# Autodesk Inventor assembly: BUMP_000_Bumpers
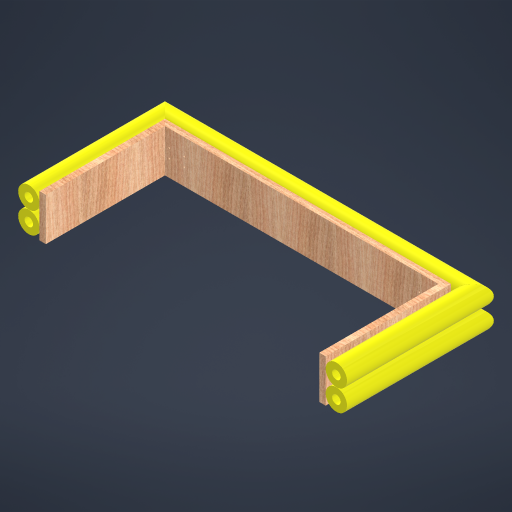
[picture p0: Inventor's stored thumbnail of the model, 512x512]
Saved by Autodesk Inventor 2024.2 (Build 282272000, 272)
## iProperties
Created: 2024-08-06
Part Number: BUMP_000_Bumpers
Document SubType Name: Assembly
Designer: Bryan
Mass: 492.361 g
Surface Area: 10037.4 cm^2
Volume: 9172.55 cm^3
Density: 0.0536776 g/cm^3
Author: Bryan
## Documents named in this file (8)
- C:\Users\bobsb\OneDrive\Documents\GitHub\1622-2024-Summer-CAD-A-Thon\Bumper\BUMP_000_Bumpers.iam
- C:\Users\bobsb\OneDrive\Documents\GitHub\1622-2024-Summer-CAD-A-Thon\Bumper\BUMP_001_Wood1.ipt
- C:\Users\bobsb\OneDrive\Documents\GitHub\1622-2024-Summer-CAD-A-Thon\Bumper\BUMP_002_Wood2.ipt
- C:\Users\bobsb\OneDrive\Documents\GitHub\1622-2024-Summer-CAD-A-Thon\COTS Library\Stucture\COTS_88805K219_Architectural 6063 Aluminum 90 Degree Angle.ipt
- C:\Users\bobsb\OneDrive\Documents\GitHub\1622-2024-Summer-CAD-A-Thon\COTS Library\Fasteners\Wood Screws\COTS_BumperWoodScrew_90031A197_Phillips Flat Head Screws for Wood.ipt
- C:\Users\bobsb\OneDrive\Documents\GitHub\1622-2024-Summer-CAD-A-Thon\Bumper\BUMP_003_Noodle1.ipt
- C:\Users\bobsb\OneDrive\Documents\GitHub\1622-2024-Summer-CAD-A-Thon\Bumper\BUMP_004_Noodle2.ipt
- C:\Users\bobsb\Downloads\th.jpg
## Components (27 placed, 6 different names)
1. BUMP_001_Wood1:1 — Mate:5, Mate:6, Flush:3, Mate:28, Mate:29, Flush:4, Mate:30, Mate:32, Mate:34, Mate:38, Mate:40, Tangent:4, Tangent:5, Angle:1
2. BUMP_002_Wood2:1 — Mate:5, Mate:6, Flush:3, Mate:33, Tangent:1, Tangent:2, Flush:6, Flush:7, Tangent:3
3. COTS_88805K219_Architectural 6063 Aluminum 90 Degree Angle:3 — Mate:32, Mate:33, Mate:36, Mate:37, Mate:39
4. COTS_88805K219_Architectural 6063 Aluminum 90 Degree Angle:4 — Mate:28, Mate:34, Mate:35, Mate:41, Mate:43
5. BUMP_002_Wood2:4 — Mate:29, Flush:4, Mate:30, Mate:35, Mate:42, Tangent:6, Tangent:7, Flush:10, Angle:2
6. BUMP_003_Noodle1:1 — Flush:5, Mate:44, Tangent:2, Flush:7, Mate:45, Mate:46
7. BUMP_004_Noodle2:1 — Mate:45, Mate:46, Tangent:5, Mate:51
8. BUMP_003_Noodle1:2 — Flush:5, Mate:44, Tangent:1, Flush:6, Tangent:3, Mate:47, Mate:48
9. BUMP_004_Noodle2:2 — Mate:47, Mate:48, Tangent:4, Mate:50, Tangent:8
10. BUMP_003_Noodle1:3 — Tangent:7, Flush:9, Mate:50, Mate:51
11. BUMP_003_Noodle1:4 — Tangent:6, Flush:9, Flush:10, Tangent:9
12. COTS_BumperWoodScrew_90031A197_Phillips Flat Head Screws for Wood:11 — Mate:36, Mate:37
13. COTS_BumperWoodScrew_90031A197_Phillips Flat Head Screws for Wood:12
14. COTS_BumperWoodScrew_90031A197_Phillips Flat Head Screws for Wood:13
15. COTS_BumperWoodScrew_90031A197_Phillips Flat Head Screws for Wood:14
16. COTS_BumperWoodScrew_90031A197_Phillips Flat Head Screws for Wood:15 — Mate:38, Mate:39
17. COTS_BumperWoodScrew_90031A197_Phillips Flat Head Screws for Wood:16
18. COTS_BumperWoodScrew_90031A197_Phillips Flat Head Screws for Wood:17
19. COTS_BumperWoodScrew_90031A197_Phillips Flat Head Screws for Wood:18
20. COTS_BumperWoodScrew_90031A197_Phillips Flat Head Screws for Wood:19 — Mate:40, Mate:41
21. COTS_BumperWoodScrew_90031A197_Phillips Flat Head Screws for Wood:20
22. COTS_BumperWoodScrew_90031A197_Phillips Flat Head Screws for Wood:21
23. COTS_BumperWoodScrew_90031A197_Phillips Flat Head Screws for Wood:22
24. COTS_BumperWoodScrew_90031A197_Phillips Flat Head Screws for Wood:23 — Mate:42, Mate:43
25. COTS_BumperWoodScrew_90031A197_Phillips Flat Head Screws for Wood:24
26. COTS_BumperWoodScrew_90031A197_Phillips Flat Head Screws for Wood:25
27. COTS_BumperWoodScrew_90031A197_Phillips Flat Head Screws for Wood:26
## Component patterns: (4 elements, first: COTS_BumperWoodScrew_90031A197_Phillips Flat Head Screws for Wood:11), (4 elements, first: COTS_BumperWoodScrew_90031A197_Phillips Flat Head Screws for Wood:15), (4 elements, first: COTS_BumperWoodScrew_90031A197_Phillips Flat Head Screws for Wood:19), (4 elements, first: COTS_BumperWoodScrew_90031A197_Phillips Flat Head Screws for Wood:23)
## Relationships (44: Mate 25, Tangent 9, Flush 8, Angle 2)
- Mate:5: BUMP_001_Wood1:1 ↔ BUMP_002_Wood2:1
- Mate:6: BUMP_001_Wood1:1 ↔ BUMP_002_Wood2:1
- Flush:3: BUMP_001_Wood1:1 ↔ BUMP_002_Wood2:1
- Mate:28: BUMP_001_Wood1:1 ↔ COTS_88805K219_Architectural 6063 Aluminum 90 Degree Angle:4
- Mate:29: BUMP_001_Wood1:1 ↔ BUMP_002_Wood2:4
- Flush:4: BUMP_001_Wood1:1 ↔ BUMP_002_Wood2:4
- Mate:30: BUMP_001_Wood1:1 ↔ BUMP_002_Wood2:4
- Mate:32: BUMP_001_Wood1:1 ↔ COTS_88805K219_Architectural 6063 Aluminum 90 Degree Angle:3
- Mate:33: BUMP_002_Wood2:1 ↔ COTS_88805K219_Architectural 6063 Aluminum 90 Degree Angle:3
- Mate:34: BUMP_001_Wood1:1 ↔ COTS_88805K219_Architectural 6063 Aluminum 90 Degree Angle:4
- Mate:35: COTS_88805K219_Architectural 6063 Aluminum 90 Degree Angle:4 ↔ BUMP_002_Wood2:4
- Mate:36: COTS_88805K219_Architectural 6063 Aluminum 90 Degree Angle:3 ↔ COTS_BumperWoodScrew_90031A197_Phillips Flat Head Screws for Wood:11
- Mate:37: COTS_88805K219_Architectural 6063 Aluminum 90 Degree Angle:3 ↔ COTS_BumperWoodScrew_90031A197_Phillips Flat Head Screws for Wood:11
- Mate:38: BUMP_001_Wood1:1 ↔ COTS_BumperWoodScrew_90031A197_Phillips Flat Head Screws for Wood:15
- Mate:39: COTS_88805K219_Architectural 6063 Aluminum 90 Degree Angle:3 ↔ COTS_BumperWoodScrew_90031A197_Phillips Flat Head Screws for Wood:15
- Mate:40: BUMP_001_Wood1:1 ↔ COTS_BumperWoodScrew_90031A197_Phillips Flat Head Screws for Wood:19
- Mate:41: COTS_88805K219_Architectural 6063 Aluminum 90 Degree Angle:4 ↔ COTS_BumperWoodScrew_90031A197_Phillips Flat Head Screws for Wood:19
- Mate:42: BUMP_002_Wood2:4 ↔ COTS_BumperWoodScrew_90031A197_Phillips Flat Head Screws for Wood:23
- Mate:43: COTS_88805K219_Architectural 6063 Aluminum 90 Degree Angle:4 ↔ COTS_BumperWoodScrew_90031A197_Phillips Flat Head Screws for Wood:23
- Flush:5: BUMP_003_Noodle1:1 ↔ BUMP_003_Noodle1:2
- Mate:44 (63.5 mm): BUMP_003_Noodle1:1 ↔ BUMP_003_Noodle1:2
- Tangent:1: BUMP_002_Wood2:1 ↔ BUMP_003_Noodle1:2
- Tangent:2: BUMP_002_Wood2:1 ↔ BUMP_003_Noodle1:1
- Flush:6: BUMP_002_Wood2:1 ↔ BUMP_003_Noodle1:2
- Flush:7: BUMP_002_Wood2:1 ↔ BUMP_003_Noodle1:1
- Tangent:3: BUMP_002_Wood2:1 ↔ BUMP_003_Noodle1:2
- Mate:45: BUMP_003_Noodle1:1 ↔ BUMP_004_Noodle2:1
- Mate:46: BUMP_003_Noodle1:1 ↔ BUMP_004_Noodle2:1
- Mate:47: BUMP_003_Noodle1:2 ↔ BUMP_004_Noodle2:2
- Mate:48: BUMP_003_Noodle1:2 ↔ BUMP_004_Noodle2:2
- Tangent:4: BUMP_001_Wood1:1 ↔ BUMP_004_Noodle2:2
- Tangent:5: BUMP_001_Wood1:1 ↔ BUMP_004_Noodle2:1
- [Flush]: BUMP_003_Noodle1:3 ↔ BUMP_003_Noodle1:4
- [Mate] (63.5 mm): BUMP_003_Noodle1:3 ↔ BUMP_003_Noodle1:4
- Tangent:6: BUMP_002_Wood2:4 ↔ BUMP_003_Noodle1:4
- Tangent:7: BUMP_002_Wood2:4 ↔ BUMP_003_Noodle1:3
- Flush:9: BUMP_003_Noodle1:3 ↔ BUMP_003_Noodle1:4
- Flush:10: BUMP_002_Wood2:4 ↔ BUMP_003_Noodle1:4
- Mate:50: BUMP_004_Noodle2:2 ↔ BUMP_003_Noodle1:3
- Mate:51: BUMP_004_Noodle2:1 ↔ BUMP_003_Noodle1:3
- Angle:1 (0 deg): BUMP_001_Wood1:1
- Tangent:8: BUMP_004_Noodle2:2
- Angle:2 (0 deg): BUMP_002_Wood2:4
- Tangent:9: BUMP_003_Noodle1:4
## Named parameters: d109_d96 = 0 mm, d110_d97 = 63.5 mm
